# Autodesk Inventor assembly: Frame_Skeleton
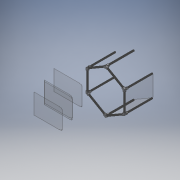
[picture p0: Inventor's stored thumbnail of the model, 180x180]
Saved by Autodesk Inventor 2019.4 (Build 234330000, 330)
## iProperties
Created: 2020-01-31
Part Number: Frame_Skeleton
Document SubType Name: Assembly
Designer: Jorian Bruslind
Author: Jorian Bruslind
## Documents named in this file (5)
- C:\Users\Jorian Bruslind\Documents\GitHub\ECE44x_Senior_Design\Design files\Delta Robot Arm\Inventor Files\Custom_Delta\Frame_Skeleton.iam
- C:\Users\Jorian Bruslind\Documents\GitHub\ECE44x_Senior_Design\Design files\Delta Robot Arm\Inventor Files\Custom_Delta\350mm_2020_tslot.ipt
- C:\Users\Jorian Bruslind\Documents\GitHub\ECE44x_Senior_Design\Design files\Delta Robot Arm\Inventor Files\Custom_Delta\60_deg_2020_joint.ipt
- C:\Users\Jorian Bruslind\Documents\GitHub\ECE44x_Senior_Design\Design files\Delta Robot Arm\Inventor Files\Custom_Delta\450mm_2020_tslot.ipt
- C:\Users\Jorian Bruslind\Documents\GitHub\ECE44x_Senior_Design\Design files\Delta Robot Arm\Inventor Files\Custom_Delta\Acrylic_Panel.ipt
## Components (24 placed, 4 different names)
1. 350mm_2020_tslot:1 — Mate:2, Mate:3, Mate:4, Mate:32, Mate:33, Mate:34, Mate:53, Mate:54
2. 350mm_2020_tslot:2 — Mate:17, Mate:18, Mate:19, Mate:20, Mate:21, Mate:22
3. 350mm_2020_tslot:3 — Mate:23, Mate:24, Mate:25, Mate:26, Mate:28, Mate:29
4. 350mm_2020_tslot:4 — Mate:5, Mate:6, Mate:7, Mate:8, Mate:9, Mate:10
5. 350mm_2020_tslot:6 — Mate:11, Mate:12, Mate:13, Mate:14, Mate:15, Mate:16
6. 60_deg_2020_joint:1 — Mate:14, Mate:15, Mate:16, Mate:17, Mate:18, Mate:19, Mate:50, Mate:51, Mate:52
7. 60_deg_2020_joint:2 — Mate:20, Mate:21, Mate:22, Mate:23, Mate:24, Mate:25, Mate:47, Mate:48, Mate:49
8. 60_deg_2020_joint:3 — Mate:1, Mate:2, Mate:3, Mate:4, Mate:5, Mate:6, Mate:7, Mate:38, Mate:39, Mate:40
9. 60_deg_2020_joint:4 — Mate:8, Mate:9, Mate:10, Mate:11, Mate:12, Mate:13, Mate:35, Mate:36, Mate:37
10. 60_deg_2020_joint:5 — Mate:32, Mate:33, Mate:34, Mate:41, Mate:42, Mate:43
11. 60_deg_2020_joint:6 — Mate:26, Mate:27, Mate:28, Mate:29, Mate:30, Mate:31, Mate:44, Mate:45, Mate:46
12. 350mm_2020_tslot:7 — Mate:27, Mate:30, Mate:31, Mate:56, Mate:57
13. 450mm_2020_tslot:1 — Mate:47, Mate:48, Mate:49
14. 450mm_2020_tslot:2 — Mate:38, Mate:39, Mate:40, Mate:55
15. 450mm_2020_tslot:3 — Mate:50, Mate:51, Mate:52
16. 450mm_2020_tslot:4 — Mate:41, Mate:42, Mate:43, Mate:58
17. 450mm_2020_tslot:5 — Mate:35, Mate:36, Mate:37
18. 450mm_2020_tslot:6 — Mate:44, Mate:45, Mate:46
19. Acrylic_Panel:1 — Mate:53, Mate:54, Mate:55
20. Acrylic_Panel:2
21. Acrylic_Panel:3 — Mate:56, Mate:57, Mate:58
22. Acrylic_Panel:4
23. Acrylic_Panel:5
24. Acrylic_Panel:6
## Relationships (58: Mate 58)
- Mate:1: 60_deg_2020_joint:3
- Mate:2: 350mm_2020_tslot:1 ↔ 60_deg_2020_joint:3
- Mate:3 (0.5 mm): 350mm_2020_tslot:1 ↔ 60_deg_2020_joint:3
- Mate:4 (0.5 mm): 350mm_2020_tslot:1 ↔ 60_deg_2020_joint:3
- Mate:5: 350mm_2020_tslot:4 ↔ 60_deg_2020_joint:3
- Mate:6 (0.5 mm): 350mm_2020_tslot:4 ↔ 60_deg_2020_joint:3
- Mate:7 (0.5 mm): 350mm_2020_tslot:4 ↔ 60_deg_2020_joint:3
- Mate:8: 350mm_2020_tslot:4 ↔ 60_deg_2020_joint:4
- Mate:9 (0.5 mm): 350mm_2020_tslot:4 ↔ 60_deg_2020_joint:4
- Mate:10 (0.5 mm): 350mm_2020_tslot:4 ↔ 60_deg_2020_joint:4
- Mate:11: 350mm_2020_tslot:6 ↔ 60_deg_2020_joint:4
- Mate:12 (0.5 mm): 350mm_2020_tslot:6 ↔ 60_deg_2020_joint:4
- Mate:13 (0.5 mm): 350mm_2020_tslot:6 ↔ 60_deg_2020_joint:4
- Mate:14: 350mm_2020_tslot:6 ↔ 60_deg_2020_joint:1
- Mate:15 (0.5 mm): 350mm_2020_tslot:6 ↔ 60_deg_2020_joint:1
- Mate:16 (0.5 mm): 350mm_2020_tslot:6 ↔ 60_deg_2020_joint:1
- Mate:17: 350mm_2020_tslot:2 ↔ 60_deg_2020_joint:1
- Mate:18 (0.5 mm): 350mm_2020_tslot:2 ↔ 60_deg_2020_joint:1
- Mate:19 (0.5 mm): 350mm_2020_tslot:2 ↔ 60_deg_2020_joint:1
- Mate:20: 350mm_2020_tslot:2 ↔ 60_deg_2020_joint:2
- Mate:21 (0.5 mm): 350mm_2020_tslot:2 ↔ 60_deg_2020_joint:2
- Mate:22 (0.5 mm): 350mm_2020_tslot:2 ↔ 60_deg_2020_joint:2
- Mate:23: 350mm_2020_tslot:3 ↔ 60_deg_2020_joint:2
- Mate:24 (0.5 mm): 350mm_2020_tslot:3 ↔ 60_deg_2020_joint:2
- Mate:25 (0.5 mm): 350mm_2020_tslot:3 ↔ 60_deg_2020_joint:2
- Mate:26: 350mm_2020_tslot:3 ↔ 60_deg_2020_joint:6
- Mate:27: 60_deg_2020_joint:6 ↔ 350mm_2020_tslot:7
- Mate:28 (0.5 mm): 350mm_2020_tslot:3 ↔ 60_deg_2020_joint:6
- Mate:29 (0.5 mm): 350mm_2020_tslot:3 ↔ 60_deg_2020_joint:6
- Mate:30 (0.5 mm): 60_deg_2020_joint:6 ↔ 350mm_2020_tslot:7
- Mate:31 (0.5 mm): 60_deg_2020_joint:6 ↔ 350mm_2020_tslot:7
- Mate:32: 350mm_2020_tslot:1 ↔ 60_deg_2020_joint:5
- Mate:33 (0.5 mm): 350mm_2020_tslot:1 ↔ 60_deg_2020_joint:5
- Mate:34 (0.5 mm): 350mm_2020_tslot:1 ↔ 60_deg_2020_joint:5
- Mate:35: 60_deg_2020_joint:4 ↔ 450mm_2020_tslot:5
- Mate:36 (0.5 mm): 60_deg_2020_joint:4 ↔ 450mm_2020_tslot:5
- Mate:37 (0.5 mm): 60_deg_2020_joint:4 ↔ 450mm_2020_tslot:5
- Mate:38: 60_deg_2020_joint:3 ↔ 450mm_2020_tslot:2
- Mate:39 (0.5 mm): 60_deg_2020_joint:3 ↔ 450mm_2020_tslot:2
- Mate:40 (0.5 mm): 60_deg_2020_joint:3 ↔ 450mm_2020_tslot:2
- Mate:41: 60_deg_2020_joint:5 ↔ 450mm_2020_tslot:4
- Mate:42 (0.5 mm): 60_deg_2020_joint:5 ↔ 450mm_2020_tslot:4
- Mate:43 (0.5 mm): 60_deg_2020_joint:5 ↔ 450mm_2020_tslot:4
- Mate:44: 60_deg_2020_joint:6 ↔ 450mm_2020_tslot:6
- Mate:45 (0.5 mm): 60_deg_2020_joint:6 ↔ 450mm_2020_tslot:6
- Mate:46 (0.5 mm): 60_deg_2020_joint:6 ↔ 450mm_2020_tslot:6
- Mate:47: 60_deg_2020_joint:2 ↔ 450mm_2020_tslot:1
- Mate:48 (0.5 mm): 60_deg_2020_joint:2 ↔ 450mm_2020_tslot:1
- Mate:49 (0.5 mm): 60_deg_2020_joint:2 ↔ 450mm_2020_tslot:1
- Mate:50: 60_deg_2020_joint:1 ↔ 450mm_2020_tslot:3
- Mate:51 (0.5 mm): 60_deg_2020_joint:1 ↔ 450mm_2020_tslot:3
- Mate:52 (0.5 mm): 60_deg_2020_joint:1 ↔ 450mm_2020_tslot:3
- Mate:53: 350mm_2020_tslot:1 ↔ Acrylic_Panel:1
- Mate:54 (0.5 mm): 350mm_2020_tslot:1 ↔ Acrylic_Panel:1
- Mate:55 (1 mm): 450mm_2020_tslot:2 ↔ Acrylic_Panel:1
- Mate:56: 350mm_2020_tslot:7 ↔ Acrylic_Panel:3
- Mate:57: 350mm_2020_tslot:7 ↔ Acrylic_Panel:3
- Mate:58 (1 mm): 450mm_2020_tslot:4 ↔ Acrylic_Panel:3
